# Autodesk Inventor assembly: face
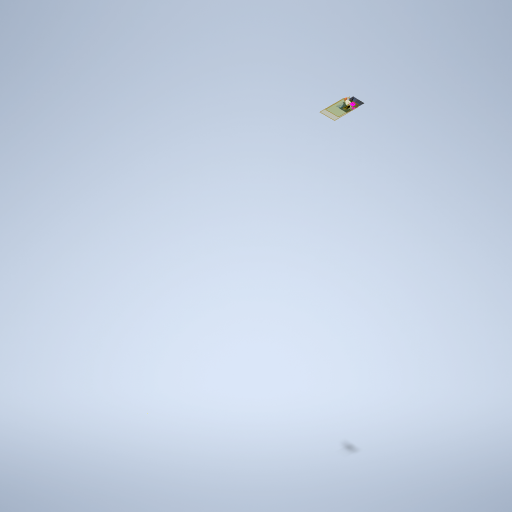
[picture p0: Inventor's stored thumbnail of the model, 512x512]
Saved by Autodesk Inventor 2023.2 (Build 272271030, 271C)
## iProperties
Created: 2024-01-26
Part Number: face
Document SubType Name: Assembly
Designer: I9232
Author: I9232
## Documents named in this file (37)
- D:\!project\fox_n_crow_construction\crow\face\face.iam
- D:\!project\fox_n_crow_construction\crow\face\Сборка глаза вороны.iam
- D:\!project\fox_n_crow_construction\crow\face\Деталь1.ipt
- D:\!project\fox_n_crow_construction\crow\face\Платформа для крыльев лево.ipt
- D:\!project\fox_n_crow_construction\crow\face\Платформа для крыльев право.ipt
- D:\!project\fox_n_crow_construction\crow\face\Сыр.ipt
- D:\!project\fox_n_crow_construction\crow\face\Веер.ipt
- D:\!project\fox_n_crow_construction\crow\face\боковые стороны головы.ipt
- D:\!project\fox_n_crow_construction\crow\face\servoDS3115mg.iam
- D:\!project\fox_n_crow_construction\crow\face\SERVO ARM HORN 25T ALUMINIUM\SERVO ARM HORN 25T ALUMINIUM.ipt
- D:\!project\fox_n_crow_construction\crow\face\Крепление рычага к лицу.ipt
- D:\!project\fox_n_crow_construction\crow\face\Лицо низ.ipt
- D:\!project\fox_n_crow_construction\crow\face\Лицо верх.ipt
- D:\!project\fox_n_crow_construction\crow\face\Шапка для головы вороны.ipt
- D:\!project\fox_n_crow_construction\crow\face\Крепление стрелялки.ipt
- D:\!project\fox_n_crow_construction\crow\cheese_shooter\Сборка стрелялки\Сборка стрелялки.iam
- D:\!project\fox_n_crow_construction\crow\face\клюв.ipt
- D:\!project\fox_n_crow_construction\crow\face\крепежная деталь для клюва.ipt
- D:\!project\fox_n_crow_construction\crow\face\Рычаг.ipt
- D:\!project\fox_n_crow_construction\crow\face\door_hinge_MIR.iam
- D:\!project\fox_n_crow_construction\crow\face\боковые стороны головы_MIR3.ipt
- D:\!project\fox_n_crow_construction\crow\face\Нижняя часть головы.ipt
- D:\!project\fox_n_crow_construction\crow\face\Деталь крепления механизма движения головы.ipt
- D:\!project\fox_n_crow_construction\crow\rotation_block\Povorot_mec.ipt.iam
- D:\!project\fox_n_crow_construction\crow\face\Деталь крепления механизма движения головы_MIR1.ipt
- D:\!project\fox_n_crow_construction\crow\face\Вал движения головы.ipt
- D:\!project\fox_n_crow_construction\crow\face\Крепление для крепления механизма головы.ipt
- D:\!project\fox_n_crow_construction\crow\rotation_block\User Library-Bearing KFL08.ipt
- D:\!project\fox_n_crow_construction\crow\face\Рычаг головы.ipt
- D:\!project\fox_n_crow_construction\crow\face\Шпилька.ipt
- D:\!project\fox_n_crow_construction\crow\face\Трубка.ipt
- D:\!project\fox_n_crow_construction\crow\rotation_block\SHF8_Горизонтальный_держатель_вала.ipt
- D:\!project\fox_n_crow_construction\crow\face\Фиксатор головы.ipt
- D:\!project\fox_n_crow_construction\crow\face\Вал фиксатора головы.ipt
- D:\!project\fox_n_crow_construction\crow\face\Нижняя часть головы_CPY.ipt
- D:\!project\fox_n_crow_construction\crow\face\door_hinge.ipt
- Povorot_mec.ipt
## Components (46 placed, 36 different names)
1. Сборка глаза вороны:1 [sub-assembly] — Заподлицо:1, Совмещение:39, Совмещение:129, Совмещение:145
2. Платформа глаз — Заподлицо:1, Заподлицо:4, Заподлицо:5, Заподлицо:6, Совмещение:27, Совмещение:28, Заподлицо:7, Заподлицо:8, Совмещение:39, Совмещение:53, Совмещение:80
3. Платформа для крыльев лево:1
4. Платформа для крыльев право:1 — Жесткий:1
5. Сыр:1
6. Веер:1 — Жесткий:1
7. Веер:2
8. боковые стороны головы:1 — Совмещение:40, Совмещение:64, Совмещение:65, Заподлицо:10, Совмещение:81, Совмещение:97, Совмещение:116, Совмещение:169, Совмещение:172, Совмещение:173, Совмещение:179, Совмещение:180
9. servoDS3115mg:1 [sub-assembly] — Цилиндрический:10, Совмещение:40, Совмещение:43, Совмещение:64, Совмещение:65
10. Качалка сервы — Цилиндрический:10, Совмещение:43, Цилиндрический:21, Совмещение:168
11. Лицо низ:1 — Угол:2, Совмещение:54, Совмещение:56, Совмещение:57, Совмещение:62, Совмещение:63, Совмещение:109, Совмещение:150, Цилиндрический:23, Совмещение:184, Цилиндрический:25, Совмещение:186, Совмещение:187
12. Лицо верх:1 — Заподлицо:4, Заподлицо:5, Заподлицо:6, Угол:2, Совмещение:30, Совмещение:31, Совмещение:34, Совмещение:51, Совмещение:129, Цилиндрический:22, Совмещение:182, Цилиндрический:24, Совмещение:185
13. Шапка для головы вороны:1 — Совмещение:30
14. Крепление стрелялки:1 — Совмещение:27, Совмещение:28, Совмещение:32
15. Сборка стрелялки:1 [sub-assembly] — Заподлицо:7, Совмещение:31, Совмещение:32
16. клюв:2 — Совмещение:34, Заподлицо:8, Заподлицо:9, Совмещение:52
17. Крепление рычага к лицу:1 — Совмещение:56, Совмещение:57, Совмещение:109, Цилиндрический:20
18. крепежная деталь для клюва:1 — Совмещение:54, Совмещение:60, Совмещение:62, Совмещение:63
19. крепежная деталь для клюва:2 — Совмещение:51, Заподлицо:9, Совмещение:52
20. Рычаг:1 — Цилиндрический:20, Цилиндрический:21, Совмещение:168
21. клюв:3 — Совмещение:53, Совмещение:60, Совмещение:150
22. Петля правая [sub-assembly] — Цилиндрический:24, Совмещение:185, Цилиндрический:25, Совмещение:187
23. боковые стороны головы_MIR3:1 — Заподлицо:10, Совмещение:118, Совмещение:174, Совмещение:178, Совмещение:181
24. Нижняя часть головы:1 — Совмещение:179, Совмещение:180, Совмещение:181
25. Деталь крепления механизма движения головы:1 — Совмещение:151, Совмещение:154, Совмещение:157, Симметрия:1, Совмещение:164, Совмещение:165, Совмещение:167
26. Povorot_mec.ipt:1 [sub-assembly] — Совмещение:80, Совмещение:161, Совмещение:163
27. Деталь крепления механизма движения головы_MIR1:1 — Совмещение:152, Совмещение:156, Совмещение:158, Совмещение:159, Совмещение:160, Совмещение:161, Совмещение:162, Симметрия:1, Совмещение:166
28. Вал движения головы:1 — Совмещение:81, Совмещение:97, Совмещение:98, Совмещение:99, Совмещение:115, Совмещение:117, Совмещение:151, Совмещение:152
29. Ребро позвонок — Совмещение:145, Совмещение:167
30. Крепление рычага к лицу:2 — Цилиндрический:17, Совмещение:96
31. servoDS3115mg:2 [sub-assembly] — Цилиндрический:16, Совмещение:89, Совмещение:158, Совмещение:159, Совмещение:160
32. SERVO ARM HORN 25T ALUMINIUM:2 — Цилиндрический:16, Совмещение:89, Цилиндрический:18, Совмещение:128
33. User Library-Bearing KFL08:1 — Совмещение:99, Совмещение:108, Совмещение:139, Совмещение:141, Совмещение:142, Совмещение:144, Совмещение:154
34. Рычаг головы:1 — Цилиндрический:17, Цилиндрический:18, Совмещение:96, Совмещение:128
35. Шпилька:1 — Совмещение:104, Совмещение:133, Совмещение:141
36. User Library-Bearing KFL08:2 — Совмещение:98, Совмещение:104, Совмещение:105, Совмещение:140, Совмещение:162
37. Шпилька:2 — Совмещение:105, Совмещение:108, Совмещение:134, Совмещение:142
38. Трубка:1 — Совмещение:134, Совмещение:144, Совмещение:156, Совмещение:157
39. Трубка:2 — Совмещение:133, Совмещение:139, Совмещение:140
40. SHF8_Горизонтальный_держатель_вала:1 — Совмещение:115, Совмещение:116, Совмещение:169
41. SHF8_Горизонтальный_держатель_вала:2 — Совмещение:117, Совмещение:118, Совмещение:178
42. Фиксатор головы:1 — Цилиндрический:19, Совмещение:166
43. Вал фиксатора головы:1 — Цилиндрический:19, Совмещение:164, Совмещение:165
44. User Library-Bearing KFL08:3
45. Нижняя часть головы_CPY:1 — Совмещение:172, Совмещение:173, Совмещение:174
46. door_hinge:2 — Цилиндрический:22, Совмещение:182, Цилиндрический:23, Совмещение:184, Совмещение:186
## Relationships (97: Mate 75, CylindricalJoint 11, Flush 8, WeldJoint 1, Angle 1, Symmetry 1)
- Заподлицо:1 [Flush]: Сборка глаза вороны:1 ↔ Платформа глаз
- Жесткий:1 [WeldJoint]: Платформа для крыльев право:1 ↔ Веер:1
- Заподлицо:4 [Flush]: Платформа глаз ↔ Лицо верх:1
- Заподлицо:5 [Flush]: Платформа глаз ↔ Лицо верх:1
- Заподлицо:6 [Flush]: Платформа глаз ↔ Лицо верх:1
- Угол:2 [Angle] (0 deg): Лицо низ:1 ↔ Лицо верх:1
- Совмещение:27 [Mate]: Платформа глаз ↔ Крепление стрелялки:1
- Совмещение:28 [Mate]: Платформа глаз ↔ Крепление стрелялки:1
- Совмещение:30 [Mate]: Лицо верх:1 ↔ Шапка для головы вороны:1
- Заподлицо:7 [Flush]: Платформа глаз ↔ Сборка стрелялки:1
- Совмещение:31 [Mate]: Лицо верх:1 ↔ Сборка стрелялки:1
- Совмещение:32 [Mate]: Крепление стрелялки:1 ↔ Сборка стрелялки:1
- Совмещение:34 [Mate]: Лицо верх:1 ↔ клюв:2
- Заподлицо:8 [Flush]: Платформа глаз ↔ клюв:2
- Совмещение:39 [Mate]: Сборка глаза вороны:1 ↔ Платформа глаз
- Цилиндрический:10 [CylindricalJoint]: servoDS3115mg:1 ↔ Качалка сервы
- Совмещение:40 [Mate]: боковые стороны головы:1 ↔ servoDS3115mg:1
- Совмещение:43 [Mate]: servoDS3115mg:1 ↔ Качалка сервы
- Совмещение:51 [Mate]: Лицо верх:1 ↔ крепежная деталь для клюва:2
- Заподлицо:9 [Flush]: клюв:2 ↔ крепежная деталь для клюва:2
- Совмещение:52 [Mate]: клюв:2 ↔ крепежная деталь для клюва:2
- Совмещение:53 [Mate]: Платформа глаз ↔ клюв:3
- Совмещение:54 [Mate]: Лицо низ:1 ↔ крепежная деталь для клюва:1
- Совмещение:56 [Mate]: Лицо низ:1 ↔ Крепление рычага к лицу:1
- Совмещение:57 [Mate]: Лицо низ:1 ↔ Крепление рычага к лицу:1
- Совмещение:60 [Mate]: крепежная деталь для клюва:1 ↔ клюв:3
- Совмещение:62 [Mate]: Лицо низ:1 ↔ крепежная деталь для клюва:1
- Совмещение:63 [Mate]: Лицо низ:1 ↔ крепежная деталь для клюва:1
- Совмещение:64 [Mate]: боковые стороны головы:1 ↔ servoDS3115mg:1
- Совмещение:65 [Mate]: боковые стороны головы:1 ↔ servoDS3115mg:1
- Заподлицо:10 [Flush]: боковые стороны головы:1 ↔ боковые стороны головы_MIR3:1
- Совмещение:80 [Mate]: Платформа глаз ↔ Povorot_mec.ipt:1
- Совмещение:81 [Mate]: боковые стороны головы:1 ↔ Вал движения головы:1
- Цилиндрический:16 [CylindricalJoint]: servoDS3115mg:2 ↔ SERVO ARM HORN 25T ALUMINIUM:2
- Совмещение:89 [Mate]: servoDS3115mg:2 ↔ SERVO ARM HORN 25T ALUMINIUM:2
- Цилиндрический:17 [CylindricalJoint]: Крепление рычага к лицу:2 ↔ Рычаг головы:1
- Цилиндрический:18 [CylindricalJoint]: SERVO ARM HORN 25T ALUMINIUM:2 ↔ Рычаг головы:1
- Совмещение:96 [Mate]: Крепление рычага к лицу:2 ↔ Рычаг головы:1
- Совмещение:97 [Mate]: боковые стороны головы:1 ↔ Вал движения головы:1
- Совмещение:98 [Mate]: Вал движения головы:1 ↔ User Library-Bearing KFL08:2
- Совмещение:99 [Mate]: Вал движения головы:1 ↔ User Library-Bearing KFL08:1
- Совмещение:104 [Mate]: Шпилька:1 ↔ User Library-Bearing KFL08:2
- Совмещение:105 [Mate]: User Library-Bearing KFL08:2 ↔ Шпилька:2
- Совмещение:108 [Mate]: User Library-Bearing KFL08:1 ↔ Шпилька:2
- Совмещение:109 [Mate]: Лицо низ:1 ↔ Крепление рычага к лицу:1
- Совмещение:115 [Mate]: Вал движения головы:1 ↔ SHF8_Горизонтальный_держатель_вала:1
- Совмещение:116 [Mate]: боковые стороны головы:1 ↔ SHF8_Горизонтальный_держатель_вала:1
- Совмещение:117 [Mate]: Вал движения головы:1 ↔ SHF8_Горизонтальный_держатель_вала:2
- Совмещение:118 [Mate]: боковые стороны головы_MIR3:1 ↔ SHF8_Горизонтальный_держатель_вала:2
- Цилиндрический:19 [CylindricalJoint]: Фиксатор головы:1 ↔ Вал фиксатора головы:1
- Совмещение:128 [Mate]: SERVO ARM HORN 25T ALUMINIUM:2 ↔ Рычаг головы:1
- Совмещение:129 [Mate]: Сборка глаза вороны:1 ↔ Лицо верх:1
- Совмещение:133 [Mate]: Шпилька:1 ↔ Трубка:2
- Совмещение:134 [Mate]: Шпилька:2 ↔ Трубка:1
- Совмещение:139 [Mate]: User Library-Bearing KFL08:1 ↔ Трубка:2
- Совмещение:140 [Mate]: User Library-Bearing KFL08:2 ↔ Трубка:2
- Совмещение:141 [Mate] (8.5 mm): User Library-Bearing KFL08:1 ↔ Шпилька:1
- Совмещение:142 [Mate] (8.5 mm): User Library-Bearing KFL08:1 ↔ Шпилька:2
- Совмещение:144 [Mate]: User Library-Bearing KFL08:1 ↔ Трубка:1
- Совмещение:145 [Mate]: Сборка глаза вороны:1 ↔ Ребро позвонок
- Совмещение:150 [Mate]: Лицо низ:1 ↔ клюв:3
- Совмещение:151 [Mate]: Деталь крепления механизма движения головы:1 ↔ Вал движения головы:1
- Совмещение:152 [Mate]: Деталь крепления механизма движения головы_MIR1:1 ↔ Вал движения головы:1
- Совмещение:154 [Mate]: Деталь крепления механизма движения головы:1 ↔ User Library-Bearing KFL08:1
- Совмещение:156 [Mate]: Деталь крепления механизма движения головы_MIR1:1 ↔ Трубка:1
- Совмещение:157 [Mate]: Деталь крепления механизма движения головы:1 ↔ Трубка:1
- Совмещение:158 [Mate]: Деталь крепления механизма движения головы_MIR1:1 ↔ servoDS3115mg:2
- Совмещение:159 [Mate]: Деталь крепления механизма движения головы_MIR1:1 ↔ servoDS3115mg:2
- Совмещение:160 [Mate]: Деталь крепления механизма движения головы_MIR1:1 ↔ servoDS3115mg:2
- Совмещение:161 [Mate]: Povorot_mec.ipt:1 ↔ Деталь крепления механизма движения головы_MIR1:1
- Совмещение:162 [Mate]: Деталь крепления механизма движения головы_MIR1:1 ↔ User Library-Bearing KFL08:2
- Симметрия:1 [Symmetry]: Деталь крепления механизма движения головы:1 ↔ Деталь крепления механизма движения головы_MIR1:1
- Совмещение:163 [Mate]: Povorot_mec.ipt:1
- Совмещение:164 [Mate]: Деталь крепления механизма движения головы:1 ↔ Вал фиксатора головы:1
- Совмещение:165 [Mate]: Деталь крепления механизма движения головы:1 ↔ Вал фиксатора головы:1
- Совмещение:166 [Mate] (1 mm): Деталь крепления механизма движения головы_MIR1:1 ↔ Фиксатор головы:1
- Совмещение:167 [Mate]: Деталь крепления механизма движения головы:1 ↔ Ребро позвонок
- Цилиндрический:20 [CylindricalJoint]: Крепление рычага к лицу:1 ↔ Рычаг:1
- Цилиндрический:21 [CylindricalJoint]: Качалка сервы ↔ Рычаг:1
- Совмещение:168 [Mate]: Качалка сервы ↔ Рычаг:1
- Совмещение:169 [Mate]: боковые стороны головы:1 ↔ SHF8_Горизонтальный_держатель_вала:1
- Совмещение:172 [Mate]: боковые стороны головы:1 ↔ Нижняя часть головы_CPY:1
- Совмещение:173 [Mate]: боковые стороны головы:1 ↔ Нижняя часть головы_CPY:1
- Совмещение:174 [Mate]: боковые стороны головы_MIR3:1 ↔ Нижняя часть головы_CPY:1
- Совмещение:178 [Mate]: боковые стороны головы_MIR3:1 ↔ SHF8_Горизонтальный_держатель_вала:2
- Совмещение:179 [Mate]: боковые стороны головы:1 ↔ Нижняя часть головы:1
- Совмещение:180 [Mate]: боковые стороны головы:1 ↔ Нижняя часть головы:1
- Совмещение:181 [Mate]: боковые стороны головы_MIR3:1 ↔ Нижняя часть головы:1
- Цилиндрический:22 [CylindricalJoint]: Лицо верх:1 ↔ door_hinge:2
- Совмещение:182 [Mate]: Лицо верх:1 ↔ door_hinge:2
- Цилиндрический:23 [CylindricalJoint]: Лицо низ:1 ↔ door_hinge:2
- Совмещение:184 [Mate]: Лицо низ:1 ↔ door_hinge:2
- Цилиндрический:24 [CylindricalJoint]: Лицо верх:1 ↔ Петля правая
- Совмещение:185 [Mate]: Лицо верх:1 ↔ Петля правая
- Цилиндрический:25 [CylindricalJoint]: Лицо низ:1 ↔ Петля правая
- Совмещение:186 [Mate]: Лицо низ:1 ↔ door_hinge:2
- Совмещение:187 [Mate]: Лицо низ:1 ↔ Петля правая
